# Autodesk Inventor assembly: компановка емкость
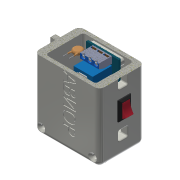
[picture p0: Inventor's stored thumbnail of the model, 180x180]
Saved by Autodesk Inventor 2021 (Build 250183000, 183)
## iProperties
Created: 2023-02-13
Part Number: компановка емкость
Document SubType Name: Assembly
Designer: Tasya
Author: Tasya
## Documents named in this file (8)
- C:\Users\Tasya\Desktop\теплица\3D\Сборки iam\компановка емкость.iam
- C:\Users\Tasya\Desktop\теплица\grabcad\Wemos_D1_mini.ipt
- C:\Users\Tasya\Desktop\теплица\grabcad\реле.ipt
- C:\Users\Tasya\Desktop\теплица\grabcad\конденсатор.ipt
- C:\Users\Tasya\Desktop\теплица\grabcad\Switch on off.ipt
- C:\Users\Tasya\Desktop\теплица\емкость\корпус емкость.ipt
- C:\Users\Tasya\Desktop\теплица\емкость\столбики.ipt
- C:\Users\Tasya\Desktop\теплица\кронштейн wemos.ipt
## Components (8 placed, 7 different names)
1. Wemos_D1_mini:1 — Совмещение:30, Заподлицо:1, Совмещение:31
2. реле:1 — Совмещение:20, Совмещение:21, Совмещение:22
3. конденсатор:1
4. Switch on off:1 — Совмещение:16, Совмещение:17, Совмещение:18
5. корпус емкость:1 — Совмещение:16, Совмещение:17, Совмещение:18, Совмещение:22, Совмещение:23, Совмещение:24, Совмещение:25, Совмещение:26
6. столбики:2 — Совмещение:23, Совмещение:26, Совмещение:27
7. столбики:1 — Совмещение:24, Совмещение:25, Совмещение:28, Совмещение:29
8. кронштейн wemos:1 — Совмещение:27, Совмещение:28, Совмещение:29, Совмещение:30, Заподлицо:1
## Relationships (16: Mate 15, Flush 1)
- Совмещение:16 [Mate]: Switch on off:1 ↔ корпус емкость:1
- Совмещение:17 [Mate]: Switch on off:1 ↔ корпус емкость:1
- Совмещение:18 [Mate] (1.7 mm): Switch on off:1 ↔ корпус емкость:1
- Совмещение:20 [Mate]: реле:1
- Совмещение:21 [Mate]: реле:1
- Совмещение:22 [Mate]: реле:1 ↔ корпус емкость:1
- Совмещение:23 [Mate]: корпус емкость:1 ↔ столбики:2
- Совмещение:24 [Mate]: корпус емкость:1 ↔ столбики:1
- Совмещение:25 [Mate]: корпус емкость:1 ↔ столбики:1
- Совмещение:26 [Mate]: корпус емкость:1 ↔ столбики:2
- Совмещение:27 [Mate]: столбики:2 ↔ кронштейн wemos:1
- Совмещение:28 [Mate]: столбики:1 ↔ кронштейн wemos:1
- Совмещение:29 [Mate]: столбики:1 ↔ кронштейн wemos:1
- Совмещение:30 [Mate]: Wemos_D1_mini:1 ↔ кронштейн wemos:1
- Заподлицо:1 [Flush]: Wemos_D1_mini:1 ↔ кронштейн wemos:1
- Совмещение:31 [Mate]: Wemos_D1_mini:1
